# Autodesk Inventor assembly: AMR
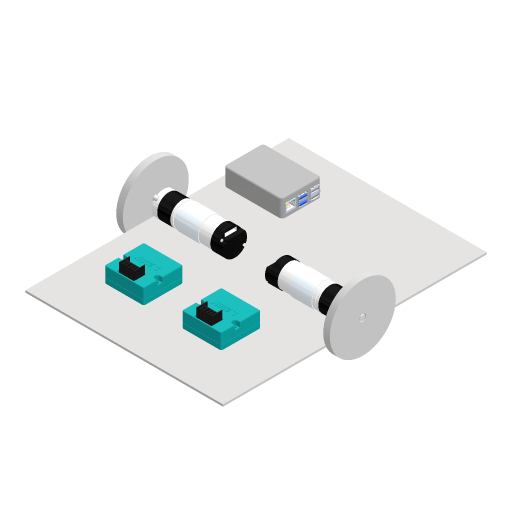
[picture p0: Inventor's stored thumbnail of the model, 512x512]
Saved by Autodesk Inventor 2024.2 (Build 282272000, 272)
## iProperties
Created: 2025-01-10
Part Number: AMR
Document SubType Name: Assembly
Designer: Kartik
Mass: 857.313 g
Surface Area: 4912.7 cm^2
Volume: 848.436 cm^3
Density: 1.01046 g/cm^3
Author: Kartik
## Documents named in this file (9)
- D:\Kartik\AMR\Basic_Robot\CAD\Assemblies\AMR.iam
- D:\Kartik\AMR\Basic_Robot\CAD\Boughtouts\Planetarygear_Motor.iam
- D:\Kartik\AMR\Basic_Robot\CAD\Parts\AMR_Base.ipt
- D:\Kartik\AMR\Basic_Robot\CAD\Parts\Wheel.ipt
- D:\Kartik\AMR\Basic_Robot\CAD\Boughtouts\h-bridge-L298n\H-brug.ipt
- D:\Kartik\AMR\Basic_Robot\CAD\Boughtouts\raspberry-pi-4-model-b\Raspberry Pi 4 Model B\Raspberry Pi 4 Model B.ipt
- D:\Kartik\AMR\Basic_Robot\CAD\Boughtouts\raspberry-pi-4-model-b-case\Raspberry_pi_4_case v2\Raspberry_pi_4_case v2.ipt
- D:\Kartik\AMR\Basic_Robot\CAD\Boughtouts\raspberry-pi-4-model-b-case\L298N Motor Driver_Cover\L298N Motor Driver_Cover.ipt
- D:\Kartik\AMR\Basic_Robot\CAD\Boughtouts\housing-motor-driver-l298n\L298N Motor Driver_Body\L298N Motor Driver_Body.ipt
## Components (13 placed, 8 different names)
1. Planetarygear_Motor:1 [sub-assembly] — Mate:1, Flush:2, Mate:4, Angle:2, Mate:5, Angle:3
2. Planetarygear_Motor:2 [sub-assembly] — Mate:2, Flush:1, Mate:5, Mate:8, Angle:4
3. AMR_Base:1 — Mate:3, Angle:1, Angle:2, Mate:6, Mate:7, Mate:8, Angle:3, Angle:4, Mate:12, Mate:19, Mate:20
4. Wheel:1 — Mate:1, Flush:2, Mate:6
5. Wheel:2 — Mate:2, Flush:1, Mate:7
6. H-brug:2 — Mate:13, Mate:14, Angle:5
7. Raspberry Pi 4 Model B:1 — Mate:10, Mate:11
8. Raspberry_pi_4_case v2:1 — Mate:10, Mate:11, Mate:12
9. L298N Motor Driver_Cover:1 — Mate:15, Flush:3, Flush:4
10. L298N Motor Driver_Body:1 — Mate:13, Mate:14, Angle:5, Mate:15, Flush:3, Flush:4, Mate:20
11. H-brug:3
12. L298N Motor Driver_Cover:2
13. L298N Motor Driver_Body:2 — Mate:19
## Relationships (31: Mate 19, Flush 6, Angle 6)
- Mate:1: Planetarygear_Motor:1 ↔ Wheel:1
- Mate:2: Planetarygear_Motor:2 ↔ Wheel:2
- Flush:1: Planetarygear_Motor:2 ↔ Wheel:2
- Flush:2: Planetarygear_Motor:1 ↔ Wheel:1
- Mate:3: AMR_Base:1
- Angle:1 (0 deg): AMR_Base:1
- Mate:4: Planetarygear_Motor:1
- Angle:2 (-90 deg): Planetarygear_Motor:1 ↔ AMR_Base:1
- Mate:5: Planetarygear_Motor:1 ↔ Planetarygear_Motor:2
- Mate:6 (2 mm): AMR_Base:1 ↔ Wheel:1
- Mate:7 (2 mm): AMR_Base:1 ↔ Wheel:2
- Mate:8 (20 mm): Planetarygear_Motor:2 ↔ AMR_Base:1
- Angle:3 (0 deg): Planetarygear_Motor:1 ↔ AMR_Base:1
- Angle:4 (0 deg): Planetarygear_Motor:2 ↔ AMR_Base:1
- Mate:10: Raspberry Pi 4 Model B:1 ↔ Raspberry_pi_4_case v2:1
- Mate:11: Raspberry Pi 4 Model B:1 ↔ Raspberry_pi_4_case v2:1
- Mate:12: AMR_Base:1 ↔ Raspberry_pi_4_case v2:1
- Mate:13: H-brug:2 ↔ L298N Motor Driver_Body:1
- Mate:14: H-brug:2 ↔ L298N Motor Driver_Body:1
- Angle:5 (0 deg): H-brug:2 ↔ L298N Motor Driver_Body:1
- Mate:15: L298N Motor Driver_Cover:1 ↔ L298N Motor Driver_Body:1
- Flush:3: L298N Motor Driver_Cover:1 ↔ L298N Motor Driver_Body:1
- Flush:4: L298N Motor Driver_Cover:1 ↔ L298N Motor Driver_Body:1
- [Mate]: H-brug:3 ↔ L298N Motor Driver_Body:2
- [Mate]: H-brug:3 ↔ L298N Motor Driver_Body:2
- [Angle] (0 deg): H-brug:3 ↔ L298N Motor Driver_Body:2
- [Mate]: L298N Motor Driver_Cover:2 ↔ L298N Motor Driver_Body:2
- [Flush]: L298N Motor Driver_Cover:2 ↔ L298N Motor Driver_Body:2
- [Flush]: L298N Motor Driver_Cover:2 ↔ L298N Motor Driver_Body:2
- Mate:19: AMR_Base:1 ↔ L298N Motor Driver_Body:2
- Mate:20: AMR_Base:1 ↔ L298N Motor Driver_Body:1
## Named parameters: d26_d20 = 0 mm, d27_d21 = 0 mm, d28_d22 = 0 deg, d29_d23 = 0 mm, d30_d24 = 0 mm, d31_d25 = 0 mm
